# Autodesk Inventor assembly: S24x1
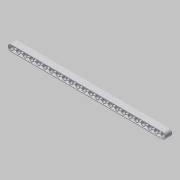
[picture p0: Inventor's stored thumbnail of the model, 180x180]
Saved by Autodesk Inventor 2019.3 (Build 233278000, 278)
## iProperties
Created: 2019-01-31
Part Number: S24x1
Document SubType Name: Assembly
Designer: Varga Daniel
Author: Varga Daniel
## Documents named in this file (11)
- C:\!_Dani\!_cloud\OneDrive\!_munka\Revolution\RevvyDemoKit\Structural parts\Beams\Straight Beams\S2+x1.iam
- C:\!_Dani\!_cloud\OneDrive\!_munka\Revolution\RevvyDemoKit\Structural parts\Beams\beam_single_end_part.ipt
- C:\!_Dani\!_cloud\OneDrive\!_munka\Revolution\RevvyDemoKit\Structural parts\Beams\beam_single_inner_part.ipt
- S12x1.iam
- S16x1.iam
- S24x1.iam
- S2x1.iam
- S3x1.iam
- S4x1.iam
- S5x1.iam
- S8x1.iam
## Components (24 placed, 2 different names)
1. beam_single_end_part:1 — Flush:1, Flush:2, Mate:1, Flush:3, Flush:4, Mate:2
2. beam_single_end_part:2 — Flush:1, Flush:2, Mate:1
3. beam_single_inner_part:1 — Flush:3, Flush:4, Mate:2
4. beam_single_inner_part:2
5. beam_single_inner_part:3
6. beam_single_inner_part:4
7. beam_single_inner_part:5
8. beam_single_inner_part:6
9. beam_single_inner_part:7
10. beam_single_inner_part:8
11. beam_single_inner_part:9
12. beam_single_inner_part:10
13. beam_single_inner_part:11
14. beam_single_inner_part:12
15. beam_single_inner_part:13
16. beam_single_inner_part:14
17. beam_single_inner_part:15
18. beam_single_inner_part:16
19. beam_single_inner_part:17
20. beam_single_inner_part:18
21. beam_single_inner_part:19
22. beam_single_inner_part:20
23. beam_single_inner_part:21
24. beam_single_inner_part:22
## Component patterns: (22 elements, first: beam_single_inner_part:1)
## Relationships (6: Flush 4, Mate 2)
- Flush:1: beam_single_end_part:1 ↔ beam_single_end_part:2
- Flush:2: beam_single_end_part:1 ↔ beam_single_end_part:2
- Mate:1 (220 mm): beam_single_end_part:1 ↔ beam_single_end_part:2
- Flush:3: beam_single_end_part:1 ↔ beam_single_inner_part:1
- Flush:4: beam_single_end_part:1 ↔ beam_single_inner_part:1
- Mate:2: beam_single_end_part:1 ↔ beam_single_inner_part:1
